# Autodesk Inventor assembly: 000.500 - Подъемная платформа
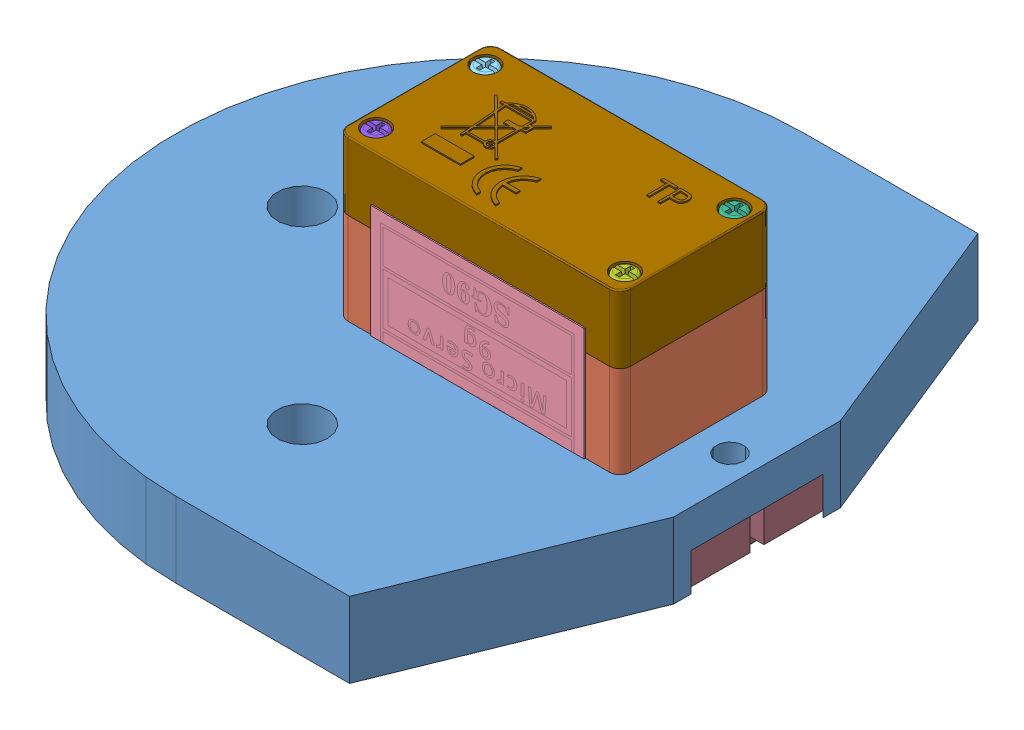
[picture p0: shaded view drawn from the shape stored in the file]
Saved by Autodesk Inventor 2019 (Build 230136000, 136)
## iProperties
Created: 2020-03-31
Part Number: 000.500 - Подъемная платформа
Material: Типовые
Document SubType Name: Assembly
Designer: Петров Иван
Author: Петров Иван
## Documents named in this file (3)
- E:\IVAN\Ivan_desktop\Kvantorium\Competitions\INOP_2020\hardware\SCARA(Dynamixels)\000.400 - Рычаг 2\000.500 - Подъемная платформа.iam
- E:\IVAN\Ivan_desktop\Kvantorium\Competitions\INOP_2020\hardware\SCARA(Dynamixels)\000.501 -  Прижим подшипников.ipt
- E:\IVAN\Ivan_desktop\Kvantorium\Competitions\INOP_2020\hardware\SCARA(Dynamixels)\components\SG90 - Micro Servo 9g - Tower Pro.1.ipt
## Components (2 placed, 2 different names)
1. 000.501 -  Прижим подшипников:1 — Совмещение:1, Совмещение:2, Совмещение:3
2. SG90 - Micro Servo 9g - Tower Pro.1:1 — Совмещение:1, Совмещение:2, Совмещение:3
## Relationships (3: Mate 3)
- Совмещение:1 [Mate]: 000.501 -  Прижим подшипников:1 ↔ SG90 - Micro Servo 9g - Tower Pro.1:1
- Совмещение:2 [Mate]: 000.501 -  Прижим подшипников:1 ↔ SG90 - Micro Servo 9g - Tower Pro.1:1
- Совмещение:3 [Mate]: 000.501 -  Прижим подшипников:1 ↔ SG90 - Micro Servo 9g - Tower Pro.1:1
